# Autodesk Inventor assembly: 4-bar intake assembly
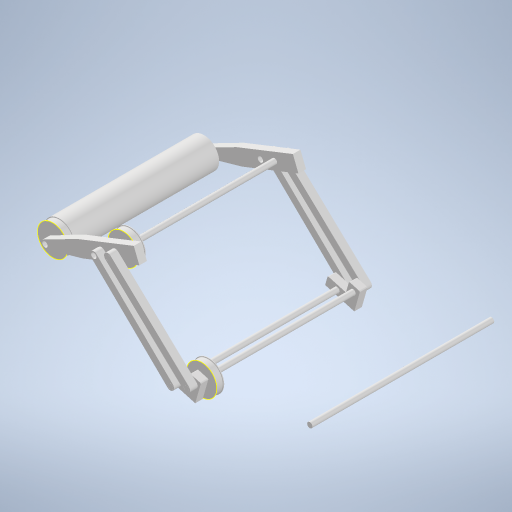
[picture p0: Inventor's stored thumbnail of the model, 512x512]
Saved by Autodesk Inventor 2023 (Build 270158030, 158C)
## iProperties
Created: 2022-07-18
Part Number: 4-bar intake assembly
Document SubType Name: Assembly
Designer: kt1040502
Author: kt1040502
## Documents named in this file (8)
- \\FRANCISTUTTLE.EDU\Home\Student\PEA\kt1040502\My Documents\4-bar intake assembly.iam
- \\FRANCISTUTTLE.EDU\Home\Student\PEA\kt1040502\My Documents\4-bar intake (14.112) bar.ipt
- \\FRANCISTUTTLE.EDU\Home\Student\PEA\kt1040502\My Documents\4-bar intake (14.258) bar.ipt
- \\FRANCISTUTTLE.EDU\Home\Student\PEA\kt1040502\My Documents\4-bar intake block.ipt
- \\FRANCISTUTTLE.EDU\Home\Student\PEA\kt1040502\My Documents\4-bar intake mount.ipt
- \\FRANCISTUTTLE.EDU\Home\Student\PEA\kt1040502\My Documents\4-bar intake roller.ipt
- \\FRANCISTUTTLE.EDU\Home\Student\PEA\kt1040502\My Documents\4-bar intake (24) shaft.ipt
- \\FRANCISTUTTLE.EDU\Home\Student\PEA\kt1040502\My Documents\4-bar intake () pully.ipt
## Components (16 placed, 7 different names)
1. 4-bar intake (14.112) bar:1 — Insert:1, Insert:3, Insert:19
2. 4-bar intake (14.258) bar:1 — Insert:2, Insert:4, Insert:6, Insert:11
3. 4-bar intake block:1 — Insert:3, Insert:4, Insert:8, Insert:9
4. 4-bar intake mount:1 — Insert:1, Insert:2, Insert:10
5. 4-bar intake (24) shaft:2 — Insert:6, Insert:18
6. 4-bar intake (24) shaft:3 — Insert:19, Insert:20
7. 4-bar intake (24) shaft:4
8. 4-bar intake (24) shaft:5 — Insert:11, Insert:17
9. 4-bar intake () pully:1 — Insert:9, Insert:12
10. 4-bar intake () pully:2 — Insert:8
11. 4-bar intake () pully:3 — Insert:10
12. 4-bar intake roller:1 — Insert:12
13. 4-bar intake (14.112) bar:2 — Insert:13, Insert:16, Insert:20
14. 4-bar intake (14.258) bar:2 — Insert:14, Insert:15, Insert:17, Insert:18
15. 4-bar intake block:2 — Insert:15, Insert:16
16. 4-bar intake mount:2 — Insert:13, Insert:14
## Relationships (18: Insert 18)
- Insert:1: 4-bar intake (14.112) bar:1 ↔ 4-bar intake mount:1
- Insert:2: 4-bar intake (14.258) bar:1 ↔ 4-bar intake mount:1
- Insert:3: 4-bar intake (14.112) bar:1 ↔ 4-bar intake block:1
- Insert:4: 4-bar intake (14.258) bar:1 ↔ 4-bar intake block:1
- Insert:6: 4-bar intake (14.258) bar:1 ↔ 4-bar intake (24) shaft:2
- Insert:8: 4-bar intake block:1 ↔ 4-bar intake () pully:2
- Insert:9: 4-bar intake block:1 ↔ 4-bar intake () pully:1
- Insert:10: 4-bar intake mount:1 ↔ 4-bar intake () pully:3
- Insert:11: 4-bar intake (14.258) bar:1 ↔ 4-bar intake (24) shaft:5
- Insert:12: 4-bar intake () pully:1 ↔ 4-bar intake roller:1
- Insert:13: 4-bar intake (14.112) bar:2 ↔ 4-bar intake mount:2
- Insert:14: 4-bar intake (14.258) bar:2 ↔ 4-bar intake mount:2
- Insert:15: 4-bar intake (14.258) bar:2 ↔ 4-bar intake block:2
- Insert:16: 4-bar intake (14.112) bar:2 ↔ 4-bar intake block:2
- Insert:17: 4-bar intake (24) shaft:5 ↔ 4-bar intake (14.258) bar:2
- Insert:18: 4-bar intake (24) shaft:2 ↔ 4-bar intake (14.258) bar:2
- Insert:19: 4-bar intake (14.112) bar:1 ↔ 4-bar intake (24) shaft:3
- Insert:20: 4-bar intake (24) shaft:3 ↔ 4-bar intake (14.112) bar:2
